# Autodesk Inventor assembly: montaj
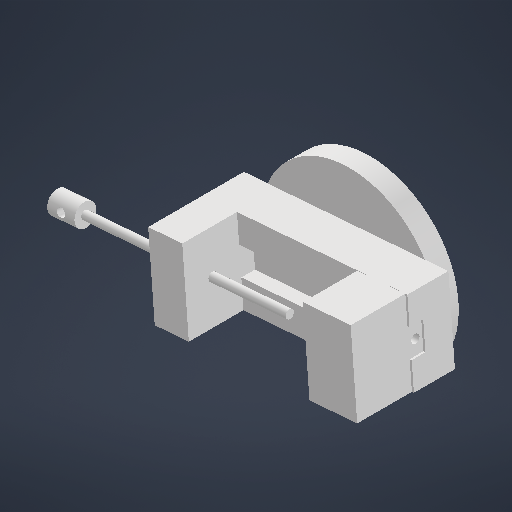
[picture p0: Inventor's stored thumbnail of the model, 512x512]
Saved by Autodesk Inventor 2025.4 (Build 294407000, 407)
## iProperties
Created: 2026-06-19
Part Number: montaj
Document SubType Name: Assembly
Designer: yigithan
Author: yigithan
## Documents named in this file (6)
- C:\Users\yigithan\Desktop\mengene\parcalar\montaj.iam
- C:\Users\yigithan\Desktop\mengene\parcalar\doner_taban.ipt
- C:\Users\yigithan\Desktop\mengene\parcalar\merkez_pimi.ipt
- C:\Users\yigithan\Desktop\mengene\parcalar\sabit_govde.ipt
- C:\Users\yigithan\Desktop\mengene\parcalar\haraketli_cene.ipt
- C:\Users\yigithan\Desktop\mengene\parcalar\ana_vida_mili.ipt
## Components (5 placed, 5 different names)
1. doner_taban:1 — Insert:1, Mate:2
2. sabit_govde:1 — Mate:1, Mate:2, Mate:3, Mate:4, Mate:5
3. merkez_pimi:2 — Insert:1, Mate:1
4. haraketli_cene:1 — Mate:3, Mate:4
5. ana_vida_mili:1 — Mate:5
## Relationships (6: Mate 5, Insert 1)
- Insert:1: doner_taban:1 ↔ merkez_pimi:2
- Mate:1: sabit_govde:1 ↔ merkez_pimi:2
- Mate:2: doner_taban:1 ↔ sabit_govde:1
- Mate:3: sabit_govde:1 ↔ haraketli_cene:1
- Mate:4: sabit_govde:1 ↔ haraketli_cene:1
- Mate:5: sabit_govde:1 ↔ ana_vida_mili:1
